# Autodesk Inventor assembly: F_TOPO
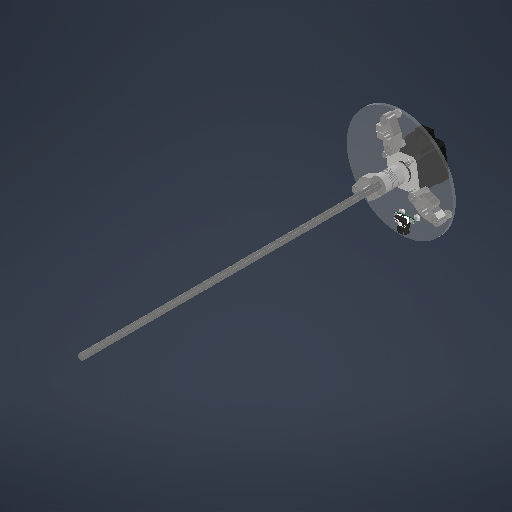
[picture p0: Inventor's stored thumbnail of the model, 512x512]
Saved by Autodesk Inventor 2025.2 (Build 292293000, 293)
## iProperties
Created: 2025-05-02
Part Number: F_TOPO
Document SubType Name: Assembly
Designer: Nelson
Author: Nelson
## Documents named in this file (14)
- C:\Users\Tiago\Documents\Inventor\Exp. Braço v1\F_TOPO.iam
- C:\Users\Tiago\Documents\Inventor\Exp. Braço v1\Topo.ipt
- C:\Users\Tiago\Documents\Inventor\Exp. Braço v1\Lead screw 2pitch_8lead_400mm.ipt
- C:\Users\Tiago\Documents\Inventor\Exp. Braço v1\NEMA17 42-38.ipt
- C:\Users\Tiago\Documents\Inventor\Exp. Braço v1\shaft_coupler 5mm_to_8mm.ipt
- C:\Users\Tiago\Documents\Inventor\Exp. Braço v1\Linear_Shaft_Support_SHF10.ipt
- C:\Users\Tiago\Documents\Inventor\Exp. Braço v1\Limit_Switch.ipt
- C:\Users\Tiago\Documents\Inventor\Exp. Braço v1\Anilha_M3.ipt
- C:\Users\Tiago\Documents\Inventor\Exp. Braço v1\M3 x0.5 ALT (...).ipt
- C:\Users\Tiago\Documents\Inventor\Exp. Braço v1\Porca_sextavada(3M).ipt
- C:\Users\Tiago\Documents\Inventor\Exp. Braço v1\M3 x8L_hexagonal_BigHEAD.ipt
- C:\Users\Tiago\Documents\Inventor\Exp. Braço v1\M5x16L_Hex.ipt
- C:\Users\Tiago\Documents\Inventor\Exp. Braço v1\M5_nylonLock_Nut.ipt
- C:\Users\Tiago\Documents\Inventor\Exp. Braço v1\M5x20L_Hex.ipt
## Components (32 placed, 13 different names)
1. Topo:1 — Mate:1, Mate:2, Mate:3, Mate:4, Mate:5, Mate:6, Mate:7, Mate:8, Mate:9, Mate:10, Mate:11, Mate:12, Mate:17, Mate:18, Mate:19, Insert:6, Mate:22, Mate:23, Mate:24, Insert:11, Insert:12, Insert:13, Insert:24, Insert:26, Insert:27, Insert:28, Insert:29, Insert:30
2. Lead screw 2pitch_8lead_400mm:1 — Mate:13, Mate:14, Mate:16, Rotation:1
3. NEMA17 42-38:1 — Mate:2, Mate:3, Mate:14, Mate:15, Mate:16, Mate:24, Angle:1
4. shaft_coupler 5mm_to_8mm:1 — Mate:13, Mate:15, Rotation:1
5. Linear_Shaft_Support_SHF10:1 — Mate:4, Mate:9, Mate:10, Insert:20, Insert:21
6. Linear_Shaft_Support_SHF10:2 — Mate:5, Mate:7, Mate:12, Insert:18, Insert:19
7. Linear_Shaft_Support_SHF10:3 — Mate:6, Mate:8, Mate:11, Insert:23, Insert:31
8. Limit_Switch:1 — Mate:17, Mate:18, Mate:19, Insert:9, Insert:10
9. Anilha_M3:1 — Insert:11, Insert:17
10. Anilha_M3:2 — Insert:12, Insert:16
11. Anilha_M3:3 — Insert:6, Insert:14
12. Anilha_M3:4 — Insert:13, Insert:15
13. M3 x0.5 ALT (...):5 — Insert:9, Mate:20
14. M3 x0.5 ALT (...):6 — Insert:10, Mate:21
15. Porca_sextavada(3M):1 — Mate:21, Mate:22
16. Porca_sextavada(3M):2 — Mate:20, Mate:23
17. M3 x8L_hexagonal_BigHEAD:1 — Insert:14
18. M3 x8L_hexagonal_BigHEAD:2 — Insert:15
19. M3 x8L_hexagonal_BigHEAD:3 — Insert:16
20. M3 x8L_hexagonal_BigHEAD:4 — Insert:17
21. M5x16L_Hex:1 — Insert:18
22. M5x16L_Hex:2 — Insert:21
23. M5x16L_Hex:3 — Insert:19
24. M5x16L_Hex:4 — Insert:20
25. M5x16L_Hex:6 — Insert:23
26. M5_nylonLock_Nut:1 — Insert:24
27. M5_nylonLock_Nut:2 — Insert:30, Angle:1
28. M5_nylonLock_Nut:3 — Insert:26
29. M5_nylonLock_Nut:4 — Insert:27
30. M5_nylonLock_Nut:5 — Insert:28
31. M5_nylonLock_Nut:6 — Insert:29
32. M5x20L_Hex:1 — Insert:31
## Relationships (48: Mate 24, Insert 22, RelateRotation 1, Angle 1)
- Mate:1: Topo:1
- Mate:2: Topo:1 ↔ NEMA17 42-38:1
- Mate:3: Topo:1 ↔ NEMA17 42-38:1
- Mate:4: Topo:1 ↔ Linear_Shaft_Support_SHF10:1
- Mate:5: Topo:1 ↔ Linear_Shaft_Support_SHF10:2
- Mate:6: Topo:1 ↔ Linear_Shaft_Support_SHF10:3
- Mate:7: Topo:1 ↔ Linear_Shaft_Support_SHF10:2
- Mate:8: Topo:1 ↔ Linear_Shaft_Support_SHF10:3
- Mate:9: Topo:1 ↔ Linear_Shaft_Support_SHF10:1
- Mate:10: Topo:1 ↔ Linear_Shaft_Support_SHF10:1
- Mate:11: Topo:1 ↔ Linear_Shaft_Support_SHF10:3
- Mate:12: Topo:1 ↔ Linear_Shaft_Support_SHF10:2
- Mate:13: Lead screw 2pitch_8lead_400mm:1 ↔ shaft_coupler 5mm_to_8mm:1
- Mate:14: Lead screw 2pitch_8lead_400mm:1 ↔ NEMA17 42-38:1
- Mate:15 (5 mm): NEMA17 42-38:1 ↔ shaft_coupler 5mm_to_8mm:1
- Mate:16 (1 mm): Lead screw 2pitch_8lead_400mm:1 ↔ NEMA17 42-38:1
- Mate:17: Topo:1 ↔ Limit_Switch:1
- Mate:18: Topo:1 ↔ Limit_Switch:1
- Mate:19: Topo:1 ↔ Limit_Switch:1
- Rotation:1 [RelateRotation] (1 ul): Lead screw 2pitch_8lead_400mm:1 ↔ shaft_coupler 5mm_to_8mm:1
- Insert:6: Topo:1 ↔ Anilha_M3:3
- Insert:9: Limit_Switch:1 ↔ M3 x0.5 ALT (...):5
- Insert:10: Limit_Switch:1 ↔ M3 x0.5 ALT (...):6
- Mate:20: M3 x0.5 ALT (...):5 ↔ Porca_sextavada(3M):2
- Mate:21: M3 x0.5 ALT (...):6 ↔ Porca_sextavada(3M):1
- Mate:22: Topo:1 ↔ Porca_sextavada(3M):1
- Mate:23: Topo:1 ↔ Porca_sextavada(3M):2
- Mate:24 (0.044 mm): Topo:1 ↔ NEMA17 42-38:1
- Insert:11: Topo:1 ↔ Anilha_M3:1
- Insert:12: Topo:1 ↔ Anilha_M3:2
- Insert:13: Topo:1 ↔ Anilha_M3:4
- Insert:14: Anilha_M3:3 ↔ M3 x8L_hexagonal_BigHEAD:1
- Insert:15: Anilha_M3:4 ↔ M3 x8L_hexagonal_BigHEAD:2
- Insert:16: Anilha_M3:2 ↔ M3 x8L_hexagonal_BigHEAD:3
- Insert:17: Anilha_M3:1 ↔ M3 x8L_hexagonal_BigHEAD:4
- Insert:18: Linear_Shaft_Support_SHF10:2 ↔ M5x16L_Hex:1
- Insert:19: Linear_Shaft_Support_SHF10:2 ↔ M5x16L_Hex:3
- Insert:20: Linear_Shaft_Support_SHF10:1 ↔ M5x16L_Hex:4
- Insert:21: Linear_Shaft_Support_SHF10:1 ↔ M5x16L_Hex:2
- Insert:23: Linear_Shaft_Support_SHF10:3 ↔ M5x16L_Hex:6
- Insert:24: Topo:1 ↔ M5_nylonLock_Nut:1
- Insert:26: Topo:1 ↔ M5_nylonLock_Nut:3
- Insert:27: Topo:1 ↔ M5_nylonLock_Nut:4
- Insert:28: Topo:1 ↔ M5_nylonLock_Nut:5
- Insert:29: Topo:1 ↔ M5_nylonLock_Nut:6
- Insert:30: Topo:1 ↔ M5_nylonLock_Nut:2
- Angle:1 (180 deg): NEMA17 42-38:1 ↔ M5_nylonLock_Nut:2
- Insert:31: Linear_Shaft_Support_SHF10:3 ↔ M5x20L_Hex:1
